# Autodesk Inventor assembly: DribblerUnit
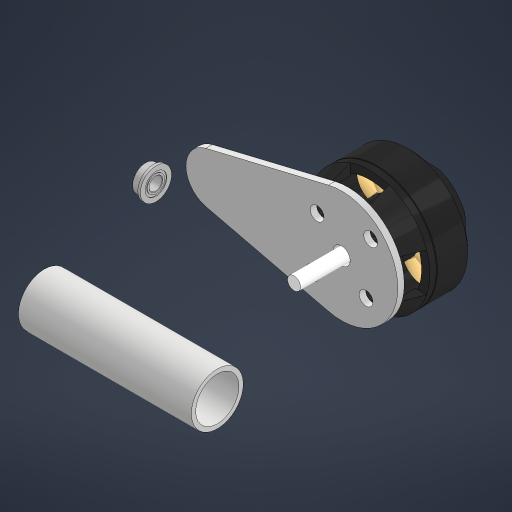
[picture p0: Inventor's stored thumbnail of the model, 512x512]
Saved by Autodesk Inventor 2024.2 (Build 282272000, 272)
## iProperties
Created: 2023-12-22
Part Number: DribblerUnit
Document SubType Name: Assembly
Designer: Hanaoka
Author: Hanaoka
## Documents named in this file (5)
- G:\共有ドライブ\reRo\05_個人\hanaoka\inventor\DribblerUnit.iam
- G:\共有ドライブ\reRo\05_個人\hanaoka\inventor\SilliconeTube_Dribbler.ipt
- G:\共有ドライブ\reRo\05_個人\hanaoka\inventor\C2822_BLDC\C2822_BLDC.ipt
- G:\共有ドライブ\reRo\05_個人\hanaoka\inventor\Dribler_main.ipt
- G:\共有ドライブ\reRo\05_個人\hanaoka\inventor\Misumi\Bearing_C-FL673ZZ\Bearing_C-FL673ZZ.ipt
## Components (4 placed, 4 different names)
1. SilliconeTube_Dribbler:1
2. C2822_BLDC:1 — フラッシュ:1
3. Dribler_main:1 — フラッシュ:1
4. Bearing_C-FL673ZZ:1
## Relationships (1: Flush 1)
- フラッシュ:1 [Flush]: C2822_BLDC:1 ↔ Dribler_main:1
